# Autodesk Inventor assembly: Sledge_Assembly
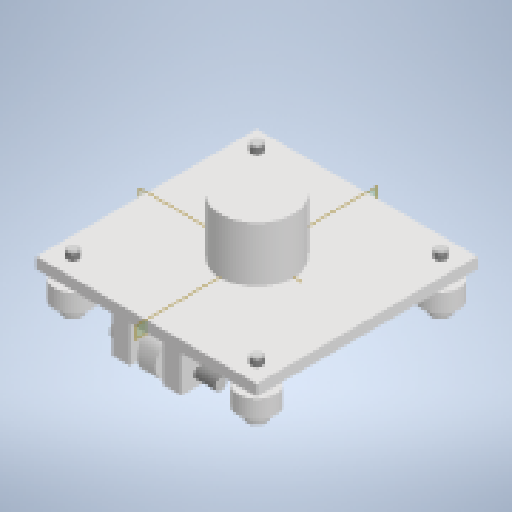
[picture p0: Inventor's stored thumbnail of the model, 512x512]
Saved by Autodesk Inventor 2025.1 (Build 291241020, 241B)
## iProperties
Created: 2024-11-07
Part Number: Sledge_Assembly
Document SubType Name: Assembly
Designer: leon-
Author: leon-
## Documents named in this file (5)
- C:\Users\leon-\OneDrive\Dokumente\Education\Berkeley\Embedded_Systems\Project\CAD Model\Sledge_Assembly.iam
- C:\Users\leon-\OneDrive\Dokumente\Education\Berkeley\Embedded_Systems\Project\CAD Model\Slege_Mounting_Plate.ipt
- C:\Users\leon-\OneDrive\Dokumente\Education\Berkeley\Embedded_Systems\Project\CAD Model\Bearing_Assembly.iam
- C:\Users\leon-\OneDrive\Dokumente\Education\Berkeley\Embedded_Systems\Project\CAD Model\Bearing_Down_Assembly.iam
- C:\Users\leon-\OneDrive\Dokumente\Education\Berkeley\Embedded_Systems\Project\CAD Model\Available_Parts\Electromagnet.ipt
## Components (8 placed, 4 different names)
1. Slege_Mounting_Plate:1 — Mate:1, Mate:2, Mate:3, Mate:4, Mate:5, Mate:6, Mate:7, Mate:8, Mate:9, Mate:10, Mate:11, Mate:12, Mate:13, Mate:14, Mate:15
2. Bearing_Assembly:1 [sub-assembly] — Mate:1, Mate:2
3. Bearing_Assembly:2 [sub-assembly] — Mate:5, Mate:8
4. Bearing_Assembly:3 [sub-assembly] — Mate:4, Mate:7
5. Bearing_Assembly:4 [sub-assembly] — Mate:3, Mate:6
6. Bearing_Down_Assembly:1 [sub-assembly] — Mate:9, Mate:11
7. Bearing_Down_Assembly:2 [sub-assembly] — Mate:10, Mate:12
8. Electromagnet:1 — Mate:13, Mate:14, Mate:15
## Relationships (15: Mate 15)
- Mate:1: Slege_Mounting_Plate:1 ↔ Bearing_Assembly:1
- Mate:2: Slege_Mounting_Plate:1 ↔ Bearing_Assembly:1
- Mate:3: Slege_Mounting_Plate:1 ↔ Bearing_Assembly:4
- Mate:4: Slege_Mounting_Plate:1 ↔ Bearing_Assembly:3
- Mate:5: Slege_Mounting_Plate:1 ↔ Bearing_Assembly:2
- Mate:6: Slege_Mounting_Plate:1 ↔ Bearing_Assembly:4
- Mate:7: Slege_Mounting_Plate:1 ↔ Bearing_Assembly:3
- Mate:8: Slege_Mounting_Plate:1 ↔ Bearing_Assembly:2
- Mate:9: Slege_Mounting_Plate:1 ↔ Bearing_Down_Assembly:1
- Mate:10: Slege_Mounting_Plate:1 ↔ Bearing_Down_Assembly:2
- Mate:11: Slege_Mounting_Plate:1 ↔ Bearing_Down_Assembly:1
- Mate:12: Slege_Mounting_Plate:1 ↔ Bearing_Down_Assembly:2
- Mate:13: Slege_Mounting_Plate:1 ↔ Electromagnet:1
- Mate:14: Slege_Mounting_Plate:1 ↔ Electromagnet:1
- Mate:15: Slege_Mounting_Plate:1 ↔ Electromagnet:1
